# Autodesk Inventor assembly: electronics-box
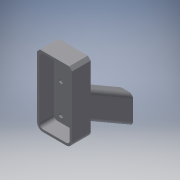
[picture p0: Inventor's stored thumbnail of the model, 180x180]
Saved by Autodesk Inventor 2017 (Build 210142000, 142)
## iProperties
Created: 2017-09-05
Part Number: electronics-box
Document SubType Name: Assembly
Designer: Hp
Author: Hp
## Documents named in this file (4)
- C:\backup\MY IMPORTANT STUFF\PROJECTS\ONGOING\POTATO GUN\electronics-box.iam
- C:\Users\Hp\Desktop\battery.ipt
- C:\Users\Hp\Desktop\handle.ipt
- C:\backup\MY IMPORTANT STUFF\PROJECTS\ONGOING\POTATO GUN\box.ipt
## Components (3 placed, 3 different names)
1. battery:1
2. handle:1 — Rotational:1
3. box:1 — Rotational:1
## Relationships (1: RevoluteJoint 1)
- Rotational:1 [RevoluteJoint]: handle:1 ↔ box:1
